# Autodesk Inventor assembly: Ensamble_carcasa_base
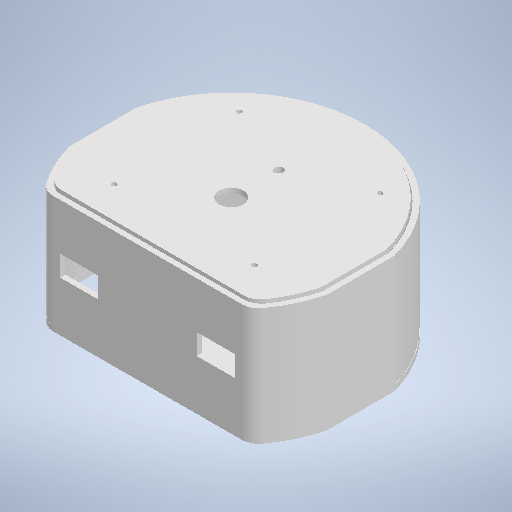
[picture p0: Inventor's stored thumbnail of the model, 512x512]
Saved by Autodesk Inventor 2025.3 (Build 293356030, 356C)
## iProperties
Created: 2025-10-16
Part Number: Ensamble_carcasa_base
Document SubType Name: Assembly
Designer: brene
Author: brene
## Documents named in this file (5)
- D:\OneDrive - Estudiantes ITCR\Documentos\GitHub\Atta-Bot-STEM\Chasis\Diseño V3.0\Ensamble_carcasa_base.iam
- D:\OneDrive - Estudiantes ITCR\Documentos\GitHub\Atta-Bot-STEM\Chasis\Diseño V3.0\base_chasis_v6\base_chasis_v4-dimsAjustadas.ipt
- D:\OneDrive - Estudiantes ITCR\Documentos\GitHub\Atta-Bot-STEM\Chasis\Rediseño_Diego&Carlos\Carcasa 4.0 Rediseño\base_chasis_v6.ipt
- D:\OneDrive - Estudiantes ITCR\Documentos\GitHub\Atta-Bot-STEM\Chasis\Diseño V3.0\carcasa4.0.ipt
- D:\OneDrive - Estudiantes ITCR\Documentos\GitHub\Atta-Bot-STEM\Chasis\Diseño V3.0\tapa_carcasa_4.0.ipt
## Components (4 placed, 3 different names)
1. base_chasis_v4-dimsAjustadas:1 — Mate:1
2. carcasa4.0:1 — Mate:1, Mate:2
3. tapa_carcasa_4.0:1
4. tapa_carcasa_4.0:2 — Mate:2
## Relationships (2: Mate 2)
- Mate:1: base_chasis_v4-dimsAjustadas:1 ↔ carcasa4.0:1
- Mate:2 (-0.847 mm): carcasa4.0:1 ↔ tapa_carcasa_4.0:2
